# Autodesk Inventor assembly: 膝_6_1
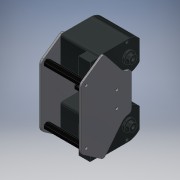
[picture p0: Inventor's stored thumbnail of the model, 180x180]
Saved by Autodesk Inventor 2018 (Build 220112000, 112)
## iProperties
Created: 2016-08-23
Part Number: 膝_6_1
Material: 一般
Document SubType Name: Assembly
Designer: hiro
Mass: 259.679 g
Surface Area: 513.454 cm^2
Volume: 137.54 cm^3
Density: 1.88802 g/cm^3
Author: hiro
## Documents named in this file (4)
- C:\Users\taka\Desktop\OPR\OpenPlatform_ver1_0\下半身_160823\膝\膝_6_1.iam
- C:\Users\taka\Desktop\OPR\OpenPlatform_ver1_0\既製品\B3M11xx.ipt
- C:\Users\taka\Desktop\OPR\OpenPlatform_ver1_0\下半身_160823\膝\膝_メインフレーム_6_1.ipt
- C:\Users\taka\Desktop\OPR\OpenPlatform_ver1_0\既製品\新規購入\AMP-340E.ipt
## Components (8 placed, 3 different names)
1. B3M11xx:1 — メイト:1, メイト:2, フラッシュ:1, 挿入:1, 挿入:2, 挿入:3, 挿入:7, 挿入:10, 挿入:11
2. 膝_メインフレーム_6_1:1 — 挿入:1, 挿入:2, 挿入:3, 挿入:4, 挿入:5, 挿入:6, 挿入:36, 挿入:37, 挿入:38, 挿入:39, 角度:1, 角度:2, 角度:3, 角度:4
3. B3M11xx:2 — 挿入:4, 挿入:5, 挿入:6, 挿入:8, 挿入:9, 挿入:12
4. 膝_メインフレーム_6_1:2 — 挿入:7, 挿入:8, 挿入:9, 挿入:10, 挿入:11, 挿入:12, 挿入:40, 挿入:41, 挿入:42, 挿入:43
5. AMP-340E:1 — 挿入:36, 挿入:43, 角度:1
6. AMP-340E:2 — 挿入:37, 挿入:42, 角度:4
7. AMP-340E:3 — 挿入:38, 挿入:40, 角度:2
8. AMP-340E:4 — 挿入:39, 挿入:41, 角度:3
## Relationships (27: Insert 20, Angle 4, Mate 2, Flush 1)
- メイト:1 [Mate] (-19.75 mm): B3M11xx:1
- メイト:2 [Mate] (-25.75 mm): B3M11xx:1
- フラッシュ:1 [Flush] (38 mm): B3M11xx:1
- 挿入:1 [Insert]: B3M11xx:1 ↔ 膝_メインフレーム_6_1:1
- 挿入:2 [Insert]: B3M11xx:1 ↔ 膝_メインフレーム_6_1:1
- 挿入:3 [Insert]: B3M11xx:1 ↔ 膝_メインフレーム_6_1:1
- 挿入:4 [Insert]: 膝_メインフレーム_6_1:1 ↔ B3M11xx:2
- 挿入:5 [Insert]: 膝_メインフレーム_6_1:1 ↔ B3M11xx:2
- 挿入:6 [Insert]: 膝_メインフレーム_6_1:1 ↔ B3M11xx:2
- 挿入:7 [Insert]: B3M11xx:1 ↔ 膝_メインフレーム_6_1:2
- 挿入:8 [Insert]: B3M11xx:2 ↔ 膝_メインフレーム_6_1:2
- 挿入:9 [Insert]: B3M11xx:2 ↔ 膝_メインフレーム_6_1:2
- 挿入:10 [Insert]: B3M11xx:1 ↔ 膝_メインフレーム_6_1:2
- 挿入:11 [Insert]: B3M11xx:1 ↔ 膝_メインフレーム_6_1:2
- 挿入:12 [Insert]: B3M11xx:2 ↔ 膝_メインフレーム_6_1:2
- 挿入:36 [Insert]: 膝_メインフレーム_6_1:1 ↔ AMP-340E:1
- 挿入:37 [Insert]: 膝_メインフレーム_6_1:1 ↔ AMP-340E:2
- 挿入:38 [Insert]: 膝_メインフレーム_6_1:1 ↔ AMP-340E:3
- 挿入:39 [Insert]: 膝_メインフレーム_6_1:1 ↔ AMP-340E:4
- 挿入:40 [Insert]: 膝_メインフレーム_6_1:2 ↔ AMP-340E:3
- 挿入:41 [Insert]: 膝_メインフレーム_6_1:2 ↔ AMP-340E:4
- 挿入:42 [Insert]: 膝_メインフレーム_6_1:2 ↔ AMP-340E:2
- 挿入:43 [Insert]: 膝_メインフレーム_6_1:2 ↔ AMP-340E:1
- 角度:1 [Angle] (0 deg): 膝_メインフレーム_6_1:1 ↔ AMP-340E:1
- 角度:2 [Angle] (0 deg): 膝_メインフレーム_6_1:1 ↔ AMP-340E:3
- 角度:3 [Angle] (0 deg): 膝_メインフレーム_6_1:1 ↔ AMP-340E:4
- 角度:4 [Angle] (0 deg): 膝_メインフレーム_6_1:1 ↔ AMP-340E:2
